# Autodesk Inventor assembly: flappy roller
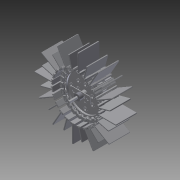
[picture p0: Inventor's stored thumbnail of the model, 180x180]
Saved by Autodesk Inventor 2014 SP1 (Build 180222100, 222)
## iProperties
Created: 2013-10-24
Part Number: flappy roller
Document SubType Name: Assembly
Designer: RyanHughes
Author: RyanHughes
## Documents named in this file (9)
- C:\Users\Ryan\Desktop\sw\toss up 2ed A bot\intake\flappy roller.iam
- C:\Users\Ryan\Desktop\sw\lib\Aperture VEX CAD Library\Sprockets\HS Sprockets\24 Tooth HS Sprocket.ipt
- C:\Users\Ryan\Desktop\sw\lib\Aperture VEX CAD Library\Tank Tread\flap-Link.ipt
- C:\Users\Ryan\Desktop\sw\lib\Aperture VEX CAD Library\Tank Tread\flaps\Conveyor-Fin-Tall.ipt
- C:\Users\Ryan\Desktop\sw\lib\Aperture VEX CAD Library\Tank Tread\flaps\Conveyor-Fin-Medium.ipt
- C:\Users\Ryan\Desktop\sw\lib\Aperture VEX CAD Library\Hardware\Shaft Collar.ipt
- C:\Users\Ryan\Desktop\sw\lib\Aperture VEX CAD Library\Spacers\SPACER-0500-0375.ipt
- C:\Users\Ryan\Desktop\sw\lib\Aperture VEX CAD Library\Shaft\3 inch Shaft.ipt
- C:\Users\Ryan\Desktop\sw\lib\Aperture VEX CAD Library\Metal\Gussets\Lockbar.ipt
## Components (54 placed, 8 different names)
1. 24 Tooth HS Sprocket:1 — Mate:1, Flush:1, Mate:2, Mate:8, Mate:9, Mate:10, Mate:13, Mate:14, Mate:15
2. Shaft Collar:1 — Mate:8, Mate:18
3. SPACER-0500-0375:1 — Mate:9, Mate:10, Mate:11, Mate:12, Flush:4
4. Shaft Collar:2 — Mate:11, Mate:12
5. 3 inch Shaft:1 — Mate:13, Mate:14, Flush:4, Mate:16, Mate:17
6. Lockbar:1 — Mate:15, Mate:16, Mate:17, Mate:18
7. Conveyor-Fin-Medium:1 — Mate:3, Mate:4, Flush:2
8. Conveyor-Fin-Tall:1 — Mate:5, Flush:3, Mate:6
9. Conveyor-Fin-Medium:2
10. Conveyor-Fin-Tall:2
11. Conveyor-Fin-Medium:3
12. Conveyor-Fin-Tall:3
13. Conveyor-Fin-Medium:4
14. Conveyor-Fin-Tall:4
15. Conveyor-Fin-Medium:5
16. Conveyor-Fin-Tall:5
17. Conveyor-Fin-Medium:6
18. Conveyor-Fin-Tall:6
19. Conveyor-Fin-Medium:7
20. Conveyor-Fin-Tall:7
21. Conveyor-Fin-Medium:8
22. Conveyor-Fin-Tall:8
23. Conveyor-Fin-Medium:9
24. Conveyor-Fin-Tall:9
25. Conveyor-Fin-Medium:10
26. Conveyor-Fin-Tall:10
27. Conveyor-Fin-Medium:11
28. Conveyor-Fin-Tall:11
29. Conveyor-Fin-Medium:12
30. Conveyor-Fin-Tall:12
31. flap-Link:1 — Mate:1, Flush:1, Mate:2, Mate:5, Flush:3, Mate:6
32. flap-Link:2 — Mate:3, Mate:4, Flush:2
33. flap-Link:3
34. flap-Link:4
35. flap-Link:5
36. flap-Link:6
37. flap-Link:7
38. flap-Link:8
39. flap-Link:9
40. flap-Link:10
41. flap-Link:11
42. flap-Link:12
43. flap-Link:13
44. flap-Link:14
45. flap-Link:15
46. flap-Link:16
47. flap-Link:17
48. flap-Link:18
49. flap-Link:19
50. flap-Link:20
51. flap-Link:21
52. flap-Link:22
53. flap-Link:23
54. flap-Link:24
## Component patterns: (12 elements, first: Conveyor-Fin-Medium:1 + Conveyor-Fin-Tall:1), (2 elements, first: flap-Link:1), Component Pattern 3:2 (2 elements), Component Pattern 3:3 (2 elements), Component Pattern 3:4 (2 elements), Component Pattern 3:5 (2 elements), Component Pattern 3:6 (2 elements), Component Pattern 3:7 (2 elements), Component Pattern 3:8 (2 elements), Component Pattern 3:9 (2 elements), Component Pattern 3:10 (2 elements), Component Pattern 3:11 (2 elements), Component Pattern 3:12 (2 elements)
## Relationships (21: Mate 17, Flush 4)
- Mate:1: 24 Tooth HS Sprocket:1 ↔ flap-Link:1
- Flush:1: 24 Tooth HS Sprocket:1 ↔ flap-Link:1
- Mate:2 (2.9845 mm): 24 Tooth HS Sprocket:1 ↔ flap-Link:1
- Mate:3: Conveyor-Fin-Medium:1 ↔ flap-Link:2
- Mate:4: Conveyor-Fin-Medium:1 ↔ flap-Link:2
- Flush:2: Conveyor-Fin-Medium:1 ↔ flap-Link:2
- Mate:5: Conveyor-Fin-Tall:1 ↔ flap-Link:1
- Flush:3: Conveyor-Fin-Tall:1 ↔ flap-Link:1
- Mate:6: Conveyor-Fin-Tall:1 ↔ flap-Link:1
- Mate:8: 24 Tooth HS Sprocket:1 ↔ Shaft Collar:1
- Mate:9: 24 Tooth HS Sprocket:1 ↔ SPACER-0500-0375:1
- Mate:10: 24 Tooth HS Sprocket:1 ↔ SPACER-0500-0375:1
- Mate:11 (7.9375 mm): SPACER-0500-0375:1 ↔ Shaft Collar:2
- Mate:12: SPACER-0500-0375:1 ↔ Shaft Collar:2
- Mate:13: 24 Tooth HS Sprocket:1 ↔ 3 inch Shaft:1
- Mate:14: 24 Tooth HS Sprocket:1 ↔ 3 inch Shaft:1
- Flush:4 (28.5242 mm): SPACER-0500-0375:1 ↔ 3 inch Shaft:1
- Mate:15: 24 Tooth HS Sprocket:1 ↔ Lockbar:1
- Mate:16: 3 inch Shaft:1 ↔ Lockbar:1
- Mate:17: 3 inch Shaft:1 ↔ Lockbar:1
- Mate:18: Shaft Collar:1 ↔ Lockbar:1
